# Autodesk Inventor assembly: Montagem2
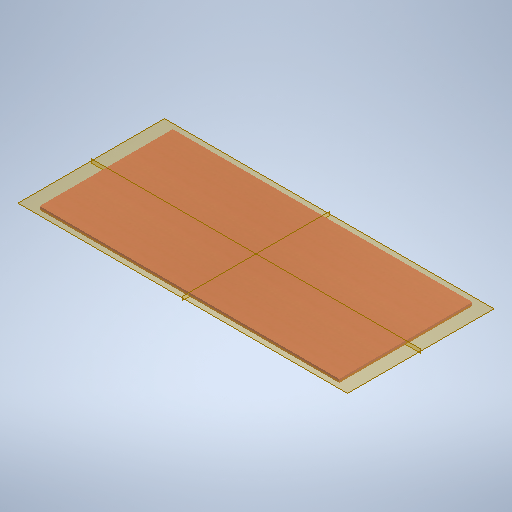
[picture p0: Inventor's stored thumbnail of the model, 512x512]
Saved by Autodesk Inventor 2025.2 (Build 292293000, 293)
## iProperties
Created: 2025-04-07
Part Number: Montagem2
Document SubType Name: Assembly
Designer: kenay
Author: kenay
## Documents named in this file (2)
- C:\Users\kenay\Documents\Aula 40horas\Montagem2.iam
- C:\Users\kenay\Documents\Aula 40horas\Peça apenas para Exercício.ipt
## Components (1 placed, 1 different names)
1. Peça apenas para Exercício:1 — Alinhado:1, Alinhado:2, Alinhado:3
## Relationships (3: Flush 3)
- Alinhado:1 [Flush]: Peça apenas para Exercício:1
- Alinhado:2 [Flush]: Peça apenas para Exercício:1
- Alinhado:3 [Flush]: Peça apenas para Exercício:1
